# Autodesk Inventor assembly: s-assy-robot
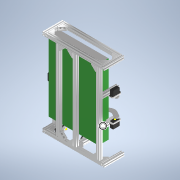
[picture p0: Inventor's stored thumbnail of the model, 180x180]
Saved by Autodesk Inventor 2022 (Build 260153000, 153)
## iProperties
Created: 2022-06-13
Part Number: s-assy-robot
Document SubType Name: Assembly
Designer: yuto6
Author: yuto6
## Documents named in this file (18)
- C:\Users\yuto6\Documents\CAD\book-reader\s-assy-robot.iam
- C:\Users\yuto6\Documents\CAD\book-reader\NFS5-2020-120.ipt
- C:\Users\yuto6\Documents\CAD\book-reader\book.ipt
- C:\Users\yuto6\Documents\CAD\book-reader\NFS5-2020-480.ipt
- C:\Users\yuto6\Documents\CAD\book-reader\NFS5-2020-330.ipt
- C:\Users\yuto6\Documents\CAD\book-reader\DCfan_normal.ipt
- C:\Users\yuto6\Documents\CAD\book-reader\s-assy-unit-motor.iam
- C:\Users\yuto6\Documents\CAD\book-reader\base2.ipt
- C:\Users\yuto6\Documents\CAD\book-reader\NFS5-2020-100.ipt
- C:\Users\yuto6\Documents\CAD\book-reader\s-assy-unit-bearing.iam
- C:\Users\yuto6\Documents\CAD\book-reader\base4.ipt
- C:\Users\yuto6\Documents\CAD\book-reader\base5.ipt
- C:\Users\yuto6\Documents\CAD\book-reader\s-assy-idler2.iam
- C:\Users\yuto6\Documents\CAD\book-reader\s-assy-idler3.iam
- C:\Users\yuto6\Documents\CAD\book-reader\belt1.ipt
- C:\Users\yuto6\Documents\CAD\book-reader\s-assy-HBLFSN5h5.iam
- C:\Users\yuto6\Documents\CAD\book-reader\s-assy-unit-motor-R.iam
- C:\Users\yuto6\Documents\CAD\book-reader\base9.ipt
## Components (44 placed, 17 different names)
1. book:1 — メイト:10
2. NFS5-2020-480:3 — メイト:3, フラッシュ:3, フラッシュ:26, メイト:39, メイト:41
3. NFS5-2020-480:4 — メイト:4, フラッシュ:4, メイト:10, フラッシュ:27, メイト:37, メイト:43, フラッシュ:31
4. NFS5-2020-480:5 — メイト:5, フラッシュ:5, メイト:45, メイト:47, フラッシュ:33, メイト:53, フラッシュ:36, メイト:54, フラッシュ:37, フラッシュ:43
5. NFS5-2020-480:6 — フラッシュ:7, メイト:6, フラッシュ:9, メイト:7, フラッシュ:10, メイト:50, メイト:52
6. DCfan_normal:1
7. s-assy-unit-motor:1 [sub-assembly] — メイト:7, フラッシュ:10, メイト:8, メイト:11, メイト:12
8. s-assy-unit-motor:2 [sub-assembly] — メイト:9, フラッシュ:11, メイト:16, メイト:18, メイト:19
9. base2:1 — メイト:11, メイト:12
10. NFS5-2020-100:1 — フラッシュ:12, メイト:13, メイト:14, メイト:15, フラッシュ:13, メイト:35
11. s-assy-unit-bearing:1 [sub-assembly] — メイト:15, フラッシュ:13, メイト:16, メイト:17, フラッシュ:14, メイト:23
12. base4:1 — メイト:17, フラッシュ:14, メイト:20, メイト:21, フラッシュ:15
13. base5:1 — メイト:18, メイト:19, メイト:20, メイト:22, フラッシュ:17
14. s-assy-idler2:1 [sub-assembly] — メイト:21, フラッシュ:15, メイト:24, メイト:25, フラッシュ:18
15. s-assy-idler3:1 [sub-assembly] — メイト:22, フラッシュ:17, フラッシュ:18
16. belt1:1 — メイト:23, メイト:24, メイト:25
17. NFS5-2020-330:3 — フラッシュ:19, フラッシュ:20, メイト:26, メイト:31, メイト:33, フラッシュ:24
18. s-assy-HBLFSN5h5:5 [sub-assembly] — メイト:33, メイト:34, フラッシュ:24
19. s-assy-HBLFSN5h5:6 [sub-assembly] — メイト:31, メイト:32, フラッシュ:23
20. s-assy-HBLFSN5h5:7 [sub-assembly] — メイト:35, メイト:36, フラッシュ:25
21. s-assy-HBLFSN5h5:8 [sub-assembly] — メイト:37, メイト:38, フラッシュ:28
22. s-assy-HBLFSN5h5:9 [sub-assembly] — メイト:39, メイト:40, フラッシュ:29
23. s-assy-HBLFSN5h5:10 [sub-assembly] — メイト:41, メイト:42, フラッシュ:30
24. s-assy-HBLFSN5h5:11 [sub-assembly] — メイト:43, メイト:44, フラッシュ:31
25. s-assy-HBLFSN5h5:12 [sub-assembly] — メイト:45, メイト:46, フラッシュ:32
26. s-assy-HBLFSN5h5:13 [sub-assembly] — メイト:47, メイト:48, フラッシュ:33
27. s-assy-HBLFSN5h5:14 [sub-assembly] — メイト:51, メイト:52, フラッシュ:35
28. s-assy-HBLFSN5h5:15 [sub-assembly] — メイト:49, メイト:50, フラッシュ:34
29. NFS5-2020-100:2 — メイト:53, フラッシュ:36, メイト:55, フラッシュ:38, メイト:56, フラッシュ:42
30. NFS5-2020-100:3 — メイト:54, フラッシュ:37, メイト:57, メイト:58, フラッシュ:39
31. s-assy-unit-motor:3 [sub-assembly] — メイト:55, フラッシュ:38, フラッシュ:40, メイト:59, メイト:60, フラッシュ:42
32. s-assy-unit-motor-R:1 [sub-assembly] — メイト:58, フラッシュ:39, フラッシュ:40, メイト:61, メイト:62
33. base9:1 — メイト:61, メイト:62, フラッシュ:41
34. base9:2 — メイト:59, メイト:60, フラッシュ:41
35. NFS5-2020-330:1 — メイト:2, フラッシュ:2, フラッシュ:12, メイト:13, メイト:28, メイト:30, メイト:36, フラッシュ:25, メイト:38, フラッシュ:28, メイト:40, フラッシュ:29, メイト:46, フラッシュ:32
36. NFS5-2020-330:2 — メイト:3, メイト:4, メイト:5, フラッシュ:3, フラッシュ:4, フラッシュ:5, フラッシュ:6, フラッシュ:19, メイト:42, フラッシュ:30, メイト:44, メイト:48
37. s-assy-HBLFSN5h5:2 [sub-assembly] — メイト:29, メイト:30, フラッシュ:22
38. s-assy-HBLFSN5h5:1 [sub-assembly] — メイト:27, フラッシュ:21, メイト:28
39. s-assy-HBLFSN5h5:3 [sub-assembly]
40. s-assy-HBLFSN5h5:4 [sub-assembly]
41. NFS5-2020-120:1 — メイト:2, フラッシュ:2, フラッシュ:9, メイト:8, メイト:9, フラッシュ:11, メイト:14, メイト:27, フラッシュ:21, フラッシュ:26, フラッシュ:27, メイト:51, フラッシュ:35
42. NFS5-2020-120:2 — フラッシュ:7, メイト:6, フラッシュ:20, メイト:26, メイト:34, メイト:49, フラッシュ:34
43. NFS5-2020-120:3 — メイト:29, フラッシュ:22, メイト:56, フラッシュ:43
44. NFS5-2020-120:4 — フラッシュ:6, メイト:32, フラッシュ:23, メイト:57
## Component patterns: (2 elements), (2 elements, first: NFS5-2020-330:1), (2 elements, first: s-assy-HBLFSN5h5:2 + s-assy-HBLFSN5h5:1), (2 elements, first: NFS5-2020-120:1), コンポーネント パターン 1:2 (2 elements)
## Relationships (101: Mate 61, Flush 40)
- メイト:2 [Mate]: NFS5-2020-330:1 ↔ NFS5-2020-120:1
- フラッシュ:2 [Flush]: NFS5-2020-330:1 ↔ NFS5-2020-120:1
- メイト:3 [Mate]: NFS5-2020-480:3 ↔ NFS5-2020-330:2
- メイト:4 [Mate]: NFS5-2020-480:4 ↔ NFS5-2020-330:2
- メイト:5 [Mate]: NFS5-2020-480:5 ↔ NFS5-2020-330:2
- フラッシュ:3 [Flush]: NFS5-2020-480:3 ↔ NFS5-2020-330:2
- フラッシュ:4 [Flush]: NFS5-2020-480:4 ↔ NFS5-2020-330:2
- フラッシュ:5 [Flush]: NFS5-2020-480:5 ↔ NFS5-2020-330:2
- フラッシュ:6 [Flush]: NFS5-2020-330:2 ↔ NFS5-2020-120:4
- フラッシュ:7 [Flush]: NFS5-2020-480:6 ↔ NFS5-2020-120:2
- メイト:6 [Mate]: NFS5-2020-480:6 ↔ NFS5-2020-120:2
- フラッシュ:9 [Flush] (-60 mm): NFS5-2020-480:6 ↔ NFS5-2020-120:1
- メイト:7 [Mate]: NFS5-2020-480:6 ↔ s-assy-unit-motor:1
- フラッシュ:10 [Flush]: NFS5-2020-480:6 ↔ s-assy-unit-motor:1
- メイト:8 [Mate] (240 mm): s-assy-unit-motor:1 ↔ NFS5-2020-120:1
- メイト:9 [Mate]: s-assy-unit-motor:2 ↔ NFS5-2020-120:1
- フラッシュ:11 [Flush]: s-assy-unit-motor:2 ↔ NFS5-2020-120:1
- メイト:10 [Mate]: book:1 ↔ NFS5-2020-480:4
- メイト:11 [Mate]: s-assy-unit-motor:1 ↔ base2:1
- メイト:12 [Mate]: s-assy-unit-motor:1 ↔ base2:1
- フラッシュ:12 [Flush]: NFS5-2020-100:1 ↔ NFS5-2020-330:1
- メイト:13 [Mate]: NFS5-2020-100:1 ↔ NFS5-2020-330:1
- メイト:14 [Mate] (150 mm): NFS5-2020-100:1 ↔ NFS5-2020-120:1
- メイト:15 [Mate]: NFS5-2020-100:1 ↔ s-assy-unit-bearing:1
- フラッシュ:13 [Flush]: NFS5-2020-100:1 ↔ s-assy-unit-bearing:1
- メイト:16 [Mate]: s-assy-unit-motor:2 ↔ s-assy-unit-bearing:1
- メイト:17 [Mate]: s-assy-unit-bearing:1 ↔ base4:1
- フラッシュ:14 [Flush]: s-assy-unit-bearing:1 ↔ base4:1
- メイト:18 [Mate]: s-assy-unit-motor:2 ↔ base5:1
- メイト:19 [Mate]: s-assy-unit-motor:2 ↔ base5:1
- メイト:20 [Mate]: base4:1 ↔ base5:1
- メイト:21 [Mate]: base4:1 ↔ s-assy-idler2:1
- フラッシュ:15 [Flush]: base4:1 ↔ s-assy-idler2:1
- メイト:22 [Mate]: base5:1 ↔ s-assy-idler3:1
- フラッシュ:17 [Flush]: base5:1 ↔ s-assy-idler3:1
- メイト:23 [Mate]: s-assy-unit-bearing:1 ↔ belt1:1
- メイト:24 [Mate]: s-assy-idler2:1 ↔ belt1:1
- メイト:25 [Mate] (1 mm): s-assy-idler2:1 ↔ belt1:1
- フラッシュ:18 [Flush]: s-assy-idler2:1 ↔ s-assy-idler3:1
- フラッシュ:19 [Flush]: NFS5-2020-330:3 ↔ NFS5-2020-330:2
- フラッシュ:20 [Flush]: NFS5-2020-330:3 ↔ NFS5-2020-120:2
- メイト:26 [Mate]: NFS5-2020-330:3 ↔ NFS5-2020-120:2
- メイト:27 [Mate]: s-assy-HBLFSN5h5:1 ↔ NFS5-2020-120:1
- フラッシュ:21 [Flush]: s-assy-HBLFSN5h5:1 ↔ NFS5-2020-120:1
- メイト:28 [Mate]: NFS5-2020-330:1 ↔ s-assy-HBLFSN5h5:1
- メイト:29 [Mate]: s-assy-HBLFSN5h5:2 ↔ NFS5-2020-120:3
- メイト:30 [Mate]: NFS5-2020-330:1 ↔ s-assy-HBLFSN5h5:2
- フラッシュ:22 [Flush]: s-assy-HBLFSN5h5:2 ↔ NFS5-2020-120:3
- メイト:31 [Mate]: NFS5-2020-330:3 ↔ s-assy-HBLFSN5h5:6
- メイト:32 [Mate]: s-assy-HBLFSN5h5:6 ↔ NFS5-2020-120:4
- フラッシュ:23 [Flush]: s-assy-HBLFSN5h5:6 ↔ NFS5-2020-120:4
- メイト:33 [Mate]: NFS5-2020-330:3 ↔ s-assy-HBLFSN5h5:5
- メイト:34 [Mate]: s-assy-HBLFSN5h5:5 ↔ NFS5-2020-120:2
- フラッシュ:24 [Flush]: NFS5-2020-330:3 ↔ s-assy-HBLFSN5h5:5
- メイト:35 [Mate]: NFS5-2020-100:1 ↔ s-assy-HBLFSN5h5:7
- メイト:36 [Mate]: s-assy-HBLFSN5h5:7 ↔ NFS5-2020-330:1
- フラッシュ:25 [Flush]: s-assy-HBLFSN5h5:7 ↔ NFS5-2020-330:1
- フラッシュ:26 [Flush] (-80 mm): NFS5-2020-480:3 ↔ NFS5-2020-120:1
- フラッシュ:27 [Flush] (-180 mm): NFS5-2020-480:4 ↔ NFS5-2020-120:1
- メイト:37 [Mate]: NFS5-2020-480:4 ↔ s-assy-HBLFSN5h5:8
- メイト:38 [Mate]: s-assy-HBLFSN5h5:8 ↔ NFS5-2020-330:1
- フラッシュ:28 [Flush]: s-assy-HBLFSN5h5:8 ↔ NFS5-2020-330:1
- メイト:39 [Mate]: NFS5-2020-480:3 ↔ s-assy-HBLFSN5h5:9
- メイト:40 [Mate]: s-assy-HBLFSN5h5:9 ↔ NFS5-2020-330:1
- フラッシュ:29 [Flush]: s-assy-HBLFSN5h5:9 ↔ NFS5-2020-330:1
- メイト:41 [Mate]: NFS5-2020-480:3 ↔ s-assy-HBLFSN5h5:10
- メイト:42 [Mate]: s-assy-HBLFSN5h5:10 ↔ NFS5-2020-330:2
- フラッシュ:30 [Flush]: s-assy-HBLFSN5h5:10 ↔ NFS5-2020-330:2
- メイト:43 [Mate]: NFS5-2020-480:4 ↔ s-assy-HBLFSN5h5:11
- メイト:44 [Mate]: s-assy-HBLFSN5h5:11 ↔ NFS5-2020-330:2
- フラッシュ:31 [Flush]: NFS5-2020-480:4 ↔ s-assy-HBLFSN5h5:11
- メイト:45 [Mate]: NFS5-2020-480:5 ↔ s-assy-HBLFSN5h5:12
- メイト:46 [Mate]: s-assy-HBLFSN5h5:12 ↔ NFS5-2020-330:1
- フラッシュ:32 [Flush]: s-assy-HBLFSN5h5:12 ↔ NFS5-2020-330:1
- メイト:47 [Mate]: NFS5-2020-480:5 ↔ s-assy-HBLFSN5h5:13
- メイト:48 [Mate]: s-assy-HBLFSN5h5:13 ↔ NFS5-2020-330:2
- フラッシュ:33 [Flush]: NFS5-2020-480:5 ↔ s-assy-HBLFSN5h5:13
- メイト:49 [Mate]: s-assy-HBLFSN5h5:15 ↔ NFS5-2020-120:2
- メイト:50 [Mate]: NFS5-2020-480:6 ↔ s-assy-HBLFSN5h5:15
- フラッシュ:34 [Flush]: s-assy-HBLFSN5h5:15 ↔ NFS5-2020-120:2
- メイト:51 [Mate]: s-assy-HBLFSN5h5:14 ↔ NFS5-2020-120:1
- メイト:52 [Mate]: NFS5-2020-480:6 ↔ s-assy-HBLFSN5h5:14
- フラッシュ:35 [Flush]: s-assy-HBLFSN5h5:14 ↔ NFS5-2020-120:1
- メイト:53 [Mate]: NFS5-2020-480:5 ↔ NFS5-2020-100:2
- フラッシュ:36 [Flush]: NFS5-2020-480:5 ↔ NFS5-2020-100:2
- メイト:54 [Mate]: NFS5-2020-480:5 ↔ NFS5-2020-100:3
- フラッシュ:37 [Flush]: NFS5-2020-480:5 ↔ NFS5-2020-100:3
- メイト:55 [Mate]: NFS5-2020-100:2 ↔ s-assy-unit-motor:3
- フラッシュ:38 [Flush]: NFS5-2020-100:2 ↔ s-assy-unit-motor:3
- メイト:56 [Mate] (150 mm): NFS5-2020-100:2 ↔ NFS5-2020-120:3
- メイト:57 [Mate] (150 mm): NFS5-2020-100:3 ↔ NFS5-2020-120:4
- メイト:58 [Mate]: NFS5-2020-100:3 ↔ s-assy-unit-motor-R:1
- フラッシュ:39 [Flush]: NFS5-2020-100:3 ↔ s-assy-unit-motor-R:1
- フラッシュ:40 [Flush]: s-assy-unit-motor:3 ↔ s-assy-unit-motor-R:1
- メイト:59 [Mate]: s-assy-unit-motor:3 ↔ base9:2
- メイト:60 [Mate]: s-assy-unit-motor:3 ↔ base9:2
- メイト:61 [Mate]: s-assy-unit-motor-R:1 ↔ base9:1
- メイト:62 [Mate]: s-assy-unit-motor-R:1 ↔ base9:1
- フラッシュ:41 [Flush]: base9:1 ↔ base9:2
- フラッシュ:42 [Flush] (10 mm): NFS5-2020-100:2 ↔ s-assy-unit-motor:3
- フラッシュ:43 [Flush] (30 mm): NFS5-2020-480:5 ↔ NFS5-2020-120:3
